# Autodesk Inventor assembly: 5mm shaft coupler assy
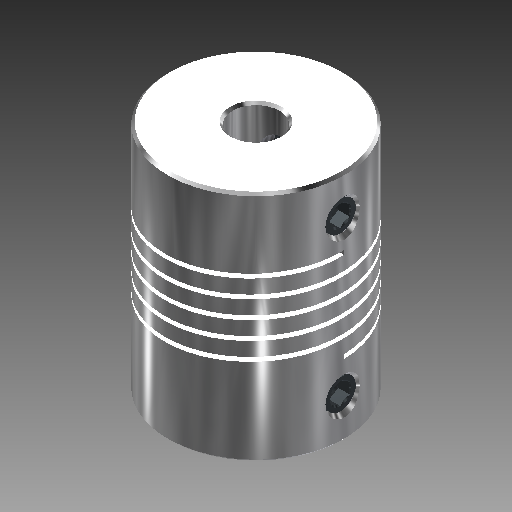
[picture p0: Inventor's stored thumbnail of the model, 512x512]
Saved by Autodesk Inventor 2018 (Build 220112000, 112)
## iProperties
Created: 2017-11-20
Part Number: 5mm shaft coupler assy
Document SubType Name: Assembly
Designer: Gabriel Smolnycki
Author: Gabriel Smolnycki
## Documents named in this file (3)
- E:\planb\mechanics\Subassemblies\5mm shaft coupler assy.iam
- E:\planb\mechanics\Hardware\5mm shaft coupler.ipt
- E:\planb\mechanics\Hardware\M4x6 Alloy SS.ipt
## Components (5 placed, 2 different names)
1. 5mm shaft coupler:1 — Insert:1, Insert:2, Insert:3, Insert:4
2. M4x6 Alloy SS:1 — Insert:4
3. M4x6 Alloy SS:2 — Insert:3
4. M4x6 Alloy SS:3 — Insert:2
5. M4x6 Alloy SS:4 — Insert:1
## Relationships (4: Insert 4)
- Insert:1: 5mm shaft coupler:1 ↔ M4x6 Alloy SS:4
- Insert:2: 5mm shaft coupler:1 ↔ M4x6 Alloy SS:3
- Insert:3: 5mm shaft coupler:1 ↔ M4x6 Alloy SS:2
- Insert:4: 5mm shaft coupler:1 ↔ M4x6 Alloy SS:1
